# Autodesk Inventor assembly: layout
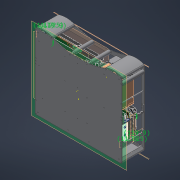
[picture p0: Inventor's stored thumbnail of the model, 180x180]
Saved by Autodesk Inventor 2022 (Build 260153000, 153)
## iProperties
Created: 2019-10-14
Part Number: layout
Material: 一般
Document SubType Name: Assembly
Designer: gisen
Author: gisen
## Documents named in this file (22)
- C:\Users\gisen\Documents\CAD\inventor\git\eatx_case\eatx_slim\layout.iam
- C:\Users\gisen\Documents\CAD\inventor\git\eatx_case\eatx_slim\resources\motherboard\Rampage V Extreme Assembly.iam
- C:\Users\gisen\Documents\CAD\inventor\git\eatx_case\eatx_slim\resources\powersupply\ATX Power Supply v1.0.iam
- C:\Users\gisen\Documents\CAD\inventor\git\eatx_case\eatx_slim\resources\gpu\ASUS TUF RTX 3070 ti.iam
- C:\Users\gisen\Documents\CAD\inventor\git\eatx_case\eatx_slim\resources\watercool\PE360.ipt
- C:\Users\gisen\Documents\CAD\inventor\git\eatx_case\eatx_slim\parts\riglt_plate_01.ipt
- C:\Users\gisen\Documents\CAD\inventor\git\eatx_case\eatx_slim\parts\left_plate_01.ipt
- C:\Users\gisen\Documents\CAD\inventor\git\eatx_case\eatx_slim\parts\SSFHRW6-130-MD4-ND4.ipt
- C:\Users\gisen\Documents\CAD\inventor\git\eatx_case\eatx_slim\parts\io_panel_adapter.ipt
- C:\Users\gisen\Documents\CAD\inventor\git\eatx_case\eatx_slim\parts\pci_slot_adapter_01.ipt
- C:\Users\gisen\Documents\CAD\inventor\git\eatx_case\eatx_slim\parts\pci_slot_adapter_02.ipt
- C:\Users\gisen\Documents\CAD\inventor\git\eatx_case\eatx_slim\parts\pci_slot_adapter_03.ipt
- C:\Users\gisen\Documents\CAD\inventor\git\eatx_case\eatx_slim\parts\pci_slot_adapter_04.ipt
- C:\Users\gisen\Documents\CAD\inventor\git\eatx_case\eatx_slim\parts\radiator_adapter_01.ipt
- C:\Users\gisen\Documents\CAD\inventor\git\eatx_case\eatx_slim\parts\power_supply_adapter_01.ipt
- C:\Users\gisen\Documents\CAD\inventor\git\eatx_case\eatx_slim\parts\gpu_supporter_01.ipt
- C:\Users\gisen\Documents\CAD\inventor\git\eatx_case\eatx_slim\parts\foot_01.ipt
- C:\Users\gisen\Documents\CAD\inventor\git\eatx_case\eatx_slim\radiator_adapter_02.ipt
- C:\Users\gisen\Documents\CAD\inventor\git\eatx_case\eatx_slim\parts\radiator_adapter_03.ipt
- C:\Users\gisen\Documents\CAD\inventor\git\eatx_case\eatx_slim\parts\left_plate_02\left_plate_02.ipt
- C:\Users\gisen\Documents\CAD\inventor\git\eatx_case\eatx_slim\parts\power_sw_plate.ipt
- C:\Users\gisen\Documents\CAD\inventor\git\eatx_case\eatx_slim\parts\power_ac_plate.ipt
## Components (47 placed, 21 different names)
1. Rampage V Extreme Assembly:1 [sub-assembly] — フラッシュ:1, メイト:7, フラッシュ:6, フラッシュ:10, 角度:1, フラッシュ:15, フラッシュ:16
2. ATX Power Supply v1.0:1 [sub-assembly] — フラッシュ:6, フラッシュ:10, フラッシュ:11, フラッシュ:32
3. ASUS TUF RTX 3070 ti:1 [sub-assembly] — メイト:7, フラッシュ:12, フラッシュ:15, フラッシュ:20, フラッシュ:25
4. PE360:1 — メイト:2, 角度:1
5. riglt_plate_01:1 — フラッシュ:2, メイト:2, メイト:8, メイト:9, メイト:10, メイト:11, メイト:12, メイト:13, メイト:14, メイト:15, メイト:16, メイト:17, メイト:18, メイト:19, メイト:20, メイト:21, メイト:22, メイト:23, メイト:24, メイト:25, メイト:26, メイト:27, メイト:29, メイト:31, メイト:33, メイト:34, メイト:35, メイト:36, メイト:37, メイト:38, フラッシュ:13, フラッシュ:17, フラッシュ:18, フラッシュ:19, メイト:41, フラッシュ:26, メイト:53, メイト:54, メイト:55, フラッシュ:31, メイト:56, メイト:62, フラッシュ:33, フラッシュ:34, メイト:66, メイト:67, メイト:68, メイト:69, フラッシュ:35
6. left_plate_01:1 — フラッシュ:5, メイト:45, メイト:46, メイト:47, メイト:60, メイト:65, メイト:70, メイト:71, メイト:72, フラッシュ:37
7. SSFHRW6-130-MD4-ND4:1 — メイト:8, メイト:18, フラッシュ:12
8. SSFHRW6-130-MD4-ND4:2 — メイト:9, メイト:19
9. SSFHRW6-130-MD4-ND4:3 — メイト:10, メイト:23, メイト:63
10. SSFHRW6-130-MD4-ND4:4 — メイト:15, メイト:26
11. SSFHRW6-130-MD4-ND4:5 — メイト:14, メイト:27
12. SSFHRW6-130-MD4-ND4:6 — メイト:13, メイト:25, フラッシュ:14, メイト:58
13. SSFHRW6-130-MD4-ND4:7 — メイト:12, メイト:24, メイト:57
14. SSFHRW6-130-MD4-ND4:8 — メイト:11, メイト:22
15. SSFHRW6-130-MD4-ND4:9 — メイト:17, メイト:20
16. SSFHRW6-130-MD4-ND4:10 — メイト:16, メイト:21, メイト:64
17. SSFHRW6-130-MD4-ND4:12 — メイト:29, メイト:31
18. SSFHRW6-130-MD4-ND4:14 — メイト:33, メイト:38, メイト:59
19. SSFHRW6-130-MD4-ND4:15 — メイト:34, メイト:37, メイト:61
20. SSFHRW6-130-MD4-ND4:16 — メイト:35, メイト:36
21. ASUS TUF RTX 3070 ti:2 [sub-assembly] — フラッシュ:13, フラッシュ:14, フラッシュ:16
22. io_panel_adapter:1 — フラッシュ:17, フラッシュ:18
23. pci_slot_adapter_01:1 — フラッシュ:19, フラッシュ:20, フラッシュ:21, フラッシュ:22, 角度:3
24. pci_slot_adapter_02:1 — フラッシュ:21, フラッシュ:22
25. pci_slot_adapter_01:2 — メイト:41, メイト:42, メイト:43, メイト:44, メイト:45, メイト:46, 角度:2
26. pci_slot_adapter_02:2 — メイト:42, メイト:43, メイト:44
27. pci_slot_adapter_03:1 — フラッシュ:25, メイト:48, メイト:75, メイト:76
28. pci_slot_adapter_04:1 — フラッシュ:26, フラッシュ:27
29. pci_slot_adapter_04:2 — メイト:47, フラッシュ:27, メイト:48
30. pci_slot_adapter_03:2 — メイト:50, メイト:51, メイト:52, フラッシュ:29, フラッシュ:30, メイト:55, メイト:73, メイト:74
31. pci_slot_adapter_04:3 — メイト:52, フラッシュ:29, メイト:53, メイト:54
32. pci_slot_adapter_04:4 — メイト:50, メイト:51, フラッシュ:30
33. radiator_adapter_01:1 — フラッシュ:31, フラッシュ:36
34. radiator_adapter_01:2 — メイト:56, メイト:57, メイト:58
35. power_supply_adapter_01:1 — フラッシュ:32
36. gpu_supporter_01:1 — メイト:59, メイト:60
37. gpu_supporter_01:2 — メイト:61, メイト:62
38. foot_01:1 — フラッシュ:33, フラッシュ:34
39. foot_01:2 — メイト:63, メイト:64, メイト:65
40. SSFHRW6-130-MD4-ND4:17 — メイト:66, メイト:67
41. SSFHRW6-130-MD4-ND4:18 — メイト:68, メイト:69
42. radiator_adapter_02:1 — フラッシュ:35
43. radiator_adapter_02:2 — メイト:70, メイト:71, メイト:72
44. radiator_adapter_03:1 — フラッシュ:36
45. left_plate_02:1 — フラッシュ:37
46. power_sw_plate:1 — メイト:73, 角度:2, メイト:74
47. power_ac_plate:1 — メイト:75, メイト:76, 角度:3
## Relationships (102: Mate 66, Flush 33, Angle 3)
- フラッシュ:1 [Flush] (5 mm): Rampage V Extreme Assembly:1
- フラッシュ:2 [Flush]: riglt_plate_01:1
- フラッシュ:4 [Flush] (-130 mm)
- メイト:2 [Mate]: PE360:1 ↔ riglt_plate_01:1
- フラッシュ:5 [Flush]: left_plate_01:1
- メイト:7 [Mate]: Rampage V Extreme Assembly:1 ↔ ASUS TUF RTX 3070 ti:1
- フラッシュ:6 [Flush]: Rampage V Extreme Assembly:1 ↔ ATX Power Supply v1.0:1
- フラッシュ:10 [Flush] (-62.22 mm): Rampage V Extreme Assembly:1 ↔ ATX Power Supply v1.0:1
- フラッシュ:11 [Flush]: ATX Power Supply v1.0:1
- 角度:1 [Angle] (180 deg): Rampage V Extreme Assembly:1 ↔ PE360:1
- メイト:8 [Mate]: riglt_plate_01:1 ↔ SSFHRW6-130-MD4-ND4:1
- メイト:9 [Mate]: riglt_plate_01:1 ↔ SSFHRW6-130-MD4-ND4:2
- メイト:10 [Mate]: riglt_plate_01:1 ↔ SSFHRW6-130-MD4-ND4:3
- メイト:11 [Mate]: riglt_plate_01:1 ↔ SSFHRW6-130-MD4-ND4:8
- メイト:12 [Mate]: riglt_plate_01:1 ↔ SSFHRW6-130-MD4-ND4:7
- メイト:13 [Mate]: riglt_plate_01:1 ↔ SSFHRW6-130-MD4-ND4:6
- メイト:14 [Mate]: riglt_plate_01:1 ↔ SSFHRW6-130-MD4-ND4:5
- メイト:15 [Mate]: riglt_plate_01:1 ↔ SSFHRW6-130-MD4-ND4:4
- メイト:16 [Mate]: riglt_plate_01:1 ↔ SSFHRW6-130-MD4-ND4:10
- メイト:17 [Mate]: riglt_plate_01:1 ↔ SSFHRW6-130-MD4-ND4:9
- メイト:18 [Mate]: riglt_plate_01:1 ↔ SSFHRW6-130-MD4-ND4:1
- メイト:19 [Mate]: riglt_plate_01:1 ↔ SSFHRW6-130-MD4-ND4:2
- メイト:20 [Mate]: riglt_plate_01:1 ↔ SSFHRW6-130-MD4-ND4:9
- メイト:21 [Mate]: riglt_plate_01:1 ↔ SSFHRW6-130-MD4-ND4:10
- メイト:22 [Mate]: riglt_plate_01:1 ↔ SSFHRW6-130-MD4-ND4:8
- メイト:23 [Mate]: riglt_plate_01:1 ↔ SSFHRW6-130-MD4-ND4:3
- メイト:24 [Mate]: riglt_plate_01:1 ↔ SSFHRW6-130-MD4-ND4:7
- メイト:25 [Mate]: riglt_plate_01:1 ↔ SSFHRW6-130-MD4-ND4:6
- メイト:26 [Mate]: riglt_plate_01:1 ↔ SSFHRW6-130-MD4-ND4:4
- メイト:27 [Mate]: riglt_plate_01:1 ↔ SSFHRW6-130-MD4-ND4:5
- メイト:29 [Mate]: riglt_plate_01:1 ↔ SSFHRW6-130-MD4-ND4:12
- メイト:31 [Mate]: riglt_plate_01:1 ↔ SSFHRW6-130-MD4-ND4:12
- メイト:33 [Mate]: riglt_plate_01:1 ↔ SSFHRW6-130-MD4-ND4:14
- メイト:34 [Mate]: riglt_plate_01:1 ↔ SSFHRW6-130-MD4-ND4:15
- メイト:35 [Mate]: riglt_plate_01:1 ↔ SSFHRW6-130-MD4-ND4:16
- メイト:36 [Mate]: riglt_plate_01:1 ↔ SSFHRW6-130-MD4-ND4:16
- メイト:37 [Mate]: riglt_plate_01:1 ↔ SSFHRW6-130-MD4-ND4:15
- メイト:38 [Mate]: riglt_plate_01:1 ↔ SSFHRW6-130-MD4-ND4:14
- フラッシュ:12 [Flush]: ASUS TUF RTX 3070 ti:1 ↔ SSFHRW6-130-MD4-ND4:1
- フラッシュ:13 [Flush] (-7.876 mm): riglt_plate_01:1 ↔ ASUS TUF RTX 3070 ti:2
- フラッシュ:14 [Flush]: SSFHRW6-130-MD4-ND4:6 ↔ ASUS TUF RTX 3070 ti:2
- フラッシュ:15 [Flush] (-10 mm): Rampage V Extreme Assembly:1 ↔ ASUS TUF RTX 3070 ti:1
- フラッシュ:16 [Flush] (-40.25 mm): Rampage V Extreme Assembly:1 ↔ ASUS TUF RTX 3070 ti:2
- フラッシュ:17 [Flush]: riglt_plate_01:1 ↔ io_panel_adapter:1
- フラッシュ:18 [Flush]: riglt_plate_01:1 ↔ io_panel_adapter:1
- フラッシュ:19 [Flush]: riglt_plate_01:1 ↔ pci_slot_adapter_01:1
- フラッシュ:20 [Flush]: ASUS TUF RTX 3070 ti:1 ↔ pci_slot_adapter_01:1
- フラッシュ:21 [Flush]: pci_slot_adapter_01:1 ↔ pci_slot_adapter_02:1
- フラッシュ:22 [Flush]: pci_slot_adapter_01:1 ↔ pci_slot_adapter_02:1
- [Flush]: pci_slot_adapter_01:2 ↔ pci_slot_adapter_02:2
- [Flush]: pci_slot_adapter_01:2 ↔ pci_slot_adapter_02:2
- メイト:41 [Mate]: riglt_plate_01:1 ↔ pci_slot_adapter_01:2
- メイト:42 [Mate]: pci_slot_adapter_01:2 ↔ pci_slot_adapter_02:2
- メイト:43 [Mate]: pci_slot_adapter_01:2 ↔ pci_slot_adapter_02:2
- メイト:44 [Mate]: pci_slot_adapter_01:2 ↔ pci_slot_adapter_02:2
- メイト:45 [Mate]: left_plate_01:1 ↔ pci_slot_adapter_01:2
- メイト:46 [Mate]: left_plate_01:1 ↔ pci_slot_adapter_01:2
- フラッシュ:25 [Flush]: ASUS TUF RTX 3070 ti:1 ↔ pci_slot_adapter_03:1
- フラッシュ:26 [Flush]: riglt_plate_01:1 ↔ pci_slot_adapter_04:1
- メイト:47 [Mate]: left_plate_01:1 ↔ pci_slot_adapter_04:2
- フラッシュ:27 [Flush]: pci_slot_adapter_04:1 ↔ pci_slot_adapter_04:2
- メイト:48 [Mate]: pci_slot_adapter_03:1 ↔ pci_slot_adapter_04:2
- [Flush]: pci_slot_adapter_04:3 ↔ pci_slot_adapter_04:4
- [Mate]: pci_slot_adapter_03:2 ↔ pci_slot_adapter_04:4
- メイト:50 [Mate]: pci_slot_adapter_03:2 ↔ pci_slot_adapter_04:4
- メイト:51 [Mate]: pci_slot_adapter_03:2 ↔ pci_slot_adapter_04:4
- メイト:52 [Mate]: pci_slot_adapter_03:2 ↔ pci_slot_adapter_04:3
- フラッシュ:29 [Flush]: pci_slot_adapter_03:2 ↔ pci_slot_adapter_04:3
- フラッシュ:30 [Flush]: pci_slot_adapter_03:2 ↔ pci_slot_adapter_04:4
- メイト:53 [Mate]: riglt_plate_01:1 ↔ pci_slot_adapter_04:3
- メイト:54 [Mate]: riglt_plate_01:1 ↔ pci_slot_adapter_04:3
- メイト:55 [Mate]: riglt_plate_01:1 ↔ pci_slot_adapter_03:2
- フラッシュ:31 [Flush]: riglt_plate_01:1 ↔ radiator_adapter_01:1
- メイト:56 [Mate]: riglt_plate_01:1 ↔ radiator_adapter_01:2
- メイト:57 [Mate]: SSFHRW6-130-MD4-ND4:7 ↔ radiator_adapter_01:2
- メイト:58 [Mate]: SSFHRW6-130-MD4-ND4:6 ↔ radiator_adapter_01:2
- フラッシュ:32 [Flush]: ATX Power Supply v1.0:1 ↔ power_supply_adapter_01:1
- メイト:59 [Mate]: SSFHRW6-130-MD4-ND4:14 ↔ gpu_supporter_01:1
- メイト:60 [Mate]: left_plate_01:1 ↔ gpu_supporter_01:1
- メイト:61 [Mate]: SSFHRW6-130-MD4-ND4:15 ↔ gpu_supporter_01:2
- メイト:62 [Mate]: riglt_plate_01:1 ↔ gpu_supporter_01:2
- フラッシュ:33 [Flush]: riglt_plate_01:1 ↔ foot_01:1
- フラッシュ:34 [Flush]: riglt_plate_01:1 ↔ foot_01:1
- メイト:63 [Mate]: SSFHRW6-130-MD4-ND4:3 ↔ foot_01:2
- メイト:64 [Mate]: SSFHRW6-130-MD4-ND4:10 ↔ foot_01:2
- メイト:65 [Mate]: left_plate_01:1 ↔ foot_01:2
- メイト:66 [Mate]: riglt_plate_01:1 ↔ SSFHRW6-130-MD4-ND4:17
- メイト:67 [Mate]: riglt_plate_01:1 ↔ SSFHRW6-130-MD4-ND4:17
- メイト:68 [Mate]: riglt_plate_01:1 ↔ SSFHRW6-130-MD4-ND4:18
- メイト:69 [Mate]: riglt_plate_01:1 ↔ SSFHRW6-130-MD4-ND4:18
- フラッシュ:35 [Flush]: riglt_plate_01:1 ↔ radiator_adapter_02:1
- メイト:70 [Mate]: left_plate_01:1 ↔ radiator_adapter_02:2
- メイト:71 [Mate]: left_plate_01:1 ↔ radiator_adapter_02:2
- メイト:72 [Mate]: left_plate_01:1 ↔ radiator_adapter_02:2
- フラッシュ:36 [Flush]: radiator_adapter_01:1 ↔ radiator_adapter_03:1
- フラッシュ:37 [Flush]: left_plate_01:1 ↔ left_plate_02:1
- メイト:73 [Mate]: pci_slot_adapter_03:2 ↔ power_sw_plate:1
- 角度:2 [Angle] (0 deg): pci_slot_adapter_01:2 ↔ power_sw_plate:1
- メイト:74 [Mate]: pci_slot_adapter_03:2 ↔ power_sw_plate:1
- メイト:75 [Mate]: pci_slot_adapter_03:1 ↔ power_ac_plate:1
- メイト:76 [Mate]: pci_slot_adapter_03:1 ↔ power_ac_plate:1
- 角度:3 [Angle] (0 deg): pci_slot_adapter_01:1 ↔ power_ac_plate:1
## Named parameters: d263_d261 = 0 mm, d264_d262 = 0 mm, d278_d276 = 0 mm, d279_d277 = 0 mm
